# Autodesk Inventor assembly: Shield Assembly
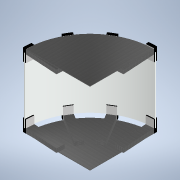
[picture p0: Inventor's stored thumbnail of the model, 180x180]
Saved by Autodesk Inventor 2020 (Build 240168000, 168)
## iProperties
Created: 2021-01-17
Part Number: Shield Assembly
Document SubType Name: Assembly
Designer: magda
Author: magda
## Documents named in this file (4)
- C:\Users\magda\OneDrive\Documents\Inventor\T3\Glock\Shield Assembly.iam
- C:\Users\magda\OneDrive\Documents\Inventor\T3\Glock\Lexan Shield.ipt
- C:\Users\magda\OneDrive\Documents\Inventor\T3\Glock\Shield Fastener.ipt
- C:\Users\magda\OneDrive\Documents\Inventor\T3\Glock\Side Shield.ipt
## Components (11 placed, 3 different names)
1. Lexan Shield:1 — Mate:1, Flush:1, Mate:2, Flush:2, Mate:3, Mate:4, Flush:3, Mate:5, Mate:6, Mate:7, Flush:4, Mate:8, Flush:5, Mate:9, Mate:10, Flush:6, Mate:11, Mate:12, Flush:7, Mate:13, Mate:14, Flush:8, Mate:15, Mate:16
2. Shield Fastener:1 — Mate:1, Flush:1, Mate:2, Mate:20, Flush:10
3. Shield Fastener:2 — Flush:2, Mate:3, Mate:4
4. Shield Fastener:3 — Flush:3, Mate:5, Mate:6
5. Shield Fastener:4 — Mate:7, Flush:4, Mate:8, Mate:19
6. Shield Fastener:5 — Flush:5, Mate:9, Mate:10, Mate:17, Flush:9
7. Shield Fastener:6 — Flush:8, Mate:15, Mate:16, Mate:18
8. Shield Fastener:7 — Flush:7, Mate:13, Mate:14
9. Shield Fastener:8 — Flush:6, Mate:11, Mate:12
10. Side Shield:1 — Mate:17, Mate:18, Flush:9
11. Side Shield:2 — Mate:19, Mate:20, Flush:10
## Relationships (30: Mate 20, Flush 10)
- Mate:1: Lexan Shield:1 ↔ Shield Fastener:1
- Flush:1: Lexan Shield:1 ↔ Shield Fastener:1
- Mate:2: Lexan Shield:1 ↔ Shield Fastener:1
- Flush:2: Lexan Shield:1 ↔ Shield Fastener:2
- Mate:3: Lexan Shield:1 ↔ Shield Fastener:2
- Mate:4: Lexan Shield:1 ↔ Shield Fastener:2
- Flush:3: Lexan Shield:1 ↔ Shield Fastener:3
- Mate:5: Lexan Shield:1 ↔ Shield Fastener:3
- Mate:6: Lexan Shield:1 ↔ Shield Fastener:3
- Mate:7: Lexan Shield:1 ↔ Shield Fastener:4
- Flush:4: Lexan Shield:1 ↔ Shield Fastener:4
- Mate:8: Lexan Shield:1 ↔ Shield Fastener:4
- Flush:5: Lexan Shield:1 ↔ Shield Fastener:5
- Mate:9: Lexan Shield:1 ↔ Shield Fastener:5
- Mate:10: Lexan Shield:1 ↔ Shield Fastener:5
- Flush:6: Lexan Shield:1 ↔ Shield Fastener:8
- Mate:11: Lexan Shield:1 ↔ Shield Fastener:8
- Mate:12: Lexan Shield:1 ↔ Shield Fastener:8
- Flush:7: Lexan Shield:1 ↔ Shield Fastener:7
- Mate:13: Lexan Shield:1 ↔ Shield Fastener:7
- Mate:14: Lexan Shield:1 ↔ Shield Fastener:7
- Flush:8: Lexan Shield:1 ↔ Shield Fastener:6
- Mate:15: Lexan Shield:1 ↔ Shield Fastener:6
- Mate:16: Lexan Shield:1 ↔ Shield Fastener:6
- Mate:17: Shield Fastener:5 ↔ Side Shield:1
- Mate:18: Shield Fastener:6 ↔ Side Shield:1
- Flush:9: Shield Fastener:5 ↔ Side Shield:1
- Mate:19: Shield Fastener:4 ↔ Side Shield:2
- Mate:20: Shield Fastener:1 ↔ Side Shield:2
- Flush:10: Shield Fastener:1 ↔ Side Shield:2
